# Autodesk Inventor assembly: HitSense
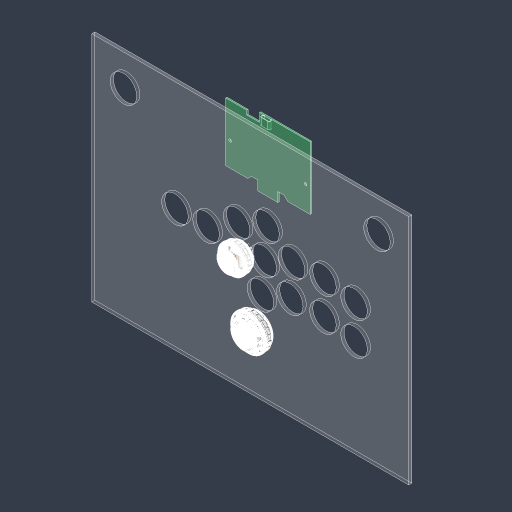
[picture p0: Inventor's stored thumbnail of the model, 512x512]
Saved by Autodesk Inventor 2023.4 (Build 274418000, 418)
## iProperties
Created: 2024-02-20
Part Number: HitSense
Document SubType Name: Assembly
Designer: JoaoSilva
Author: JoaoSilva
## Documents named in this file (10)
- C:\Users\joaos\Documents\GitHub\HitSense\CAD\HitSense.iam
- C:\Users\joaos\Documents\GitHub\HitSense\CAD\30mm_button_cap.ipt
- C:\Users\joaos\Documents\GitHub\HitSense\CAD\30mm_button_nut.ipt
- C:\Users\joaos\Documents\GitHub\HitSense\CAD\24mm_button_body.ipt
- C:\Users\joaos\Documents\GitHub\HitSense\CAD\24mm_button_cap.ipt
- C:\Users\joaos\Documents\GitHub\HitSense\CAD\24mm_button_nut.ipt
- C:\Users\joaos\Documents\GitHub\HitSense\CAD\30mm_button_body.ipt
- C:\Users\joaos\Documents\GitHub\HitSense\CAD\MX_CAD.ipt
- C:\Users\joaos\Documents\GitHub\HitSense\CAD\Top Plate Sanwa.ipt
- C:\Users\joaos\Documents\GitHub\HitSense\CAD\BDM-030.ipt
## Components (10 placed, 9 different names)
1. Top Plate Sanwa:1 — Insert:3, Insert:4, Mate:11, Flush:1, Flush:2
2. BDM-030:1 — Mate:11, Flush:1, Flush:2
3. 30mm_button_cap:1 — Mate:4, Mate:5
4. 30mm_button_nut:1 — Insert:1
5. 30mm_button_body:1 — Insert:1, Mate:1, Mate:2, Mate:3, Insert:3
6. MX_CAD:1 — Mate:1, Mate:2, Mate:3, Mate:4, Mate:5
7. 24mm_button_body:1 — Mate:6, Mate:7, Mate:8, Insert:2, Insert:4
8. 24mm_button_cap:1 — Mate:9, Mate:10
9. 24mm_button_nut:1 — Insert:2
10. MX_CAD:2 — Mate:6, Mate:7, Mate:8, Mate:9, Mate:10
## Relationships (17: Mate 11, Insert 4, Flush 2)
- Insert:1: 30mm_button_nut:1 ↔ 30mm_button_body:1
- Mate:1: 30mm_button_body:1 ↔ MX_CAD:1
- Mate:2: 30mm_button_body:1 ↔ MX_CAD:1
- Mate:3: 30mm_button_body:1 ↔ MX_CAD:1
- Mate:4: 30mm_button_cap:1 ↔ MX_CAD:1
- Mate:5: 30mm_button_cap:1 ↔ MX_CAD:1
- Mate:6: 24mm_button_body:1 ↔ MX_CAD:2
- Mate:7: 24mm_button_body:1 ↔ MX_CAD:2
- Mate:8: 24mm_button_body:1 ↔ MX_CAD:2
- Insert:2: 24mm_button_body:1 ↔ 24mm_button_nut:1
- Mate:9: 24mm_button_cap:1 ↔ MX_CAD:2
- Mate:10: 24mm_button_cap:1 ↔ MX_CAD:2
- Insert:3: Top Plate Sanwa:1 ↔ 30mm_button_body:1
- Insert:4: Top Plate Sanwa:1 ↔ 24mm_button_body:1
- Mate:11 (-18 mm): Top Plate Sanwa:1 ↔ BDM-030:1
- Flush:1: Top Plate Sanwa:1 ↔ BDM-030:1
- Flush:2 (2 mm): Top Plate Sanwa:1 ↔ BDM-030:1
